# Autodesk Inventor assembly: Robot Transporter
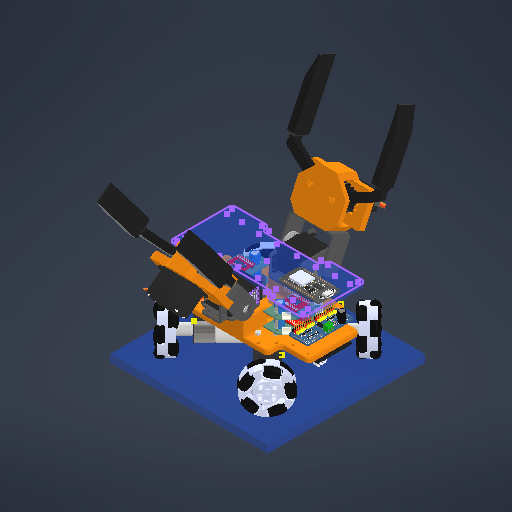
[picture p0: Inventor's stored thumbnail of the model, 512x512]
Saved by Autodesk Inventor 2026.2 (Build 302298000, 298)
## iProperties
Created: 2026-05-17
Part Number: Robot Transporter
Document SubType Name: Assembly
Designer: hando
Author: hando
## Documents named in this file (21)
- D:\Data_Lokal\Kuliah\Tri Wahyu (22518241023)\Lomba Technocorner UGM\02_Transporter\Design Robot\00_Inventor_Workspace\Robot Transporter.iam
- D:\Data_Lokal\Kuliah\Tri Wahyu (22518241023)\Lomba Technocorner UGM\02_Transporter\Design Robot\00_Inventor_Workspace\bringsmart-jga25-371-12v-dc-geared-motor-with-encoder-collection-1.snapshot.3\JGA25-371_12VDC_400RPM.ipt
- D:\Data_Lokal\Kuliah\Tri Wahyu (22518241023)\Lomba Technocorner UGM\02_Transporter\Design Robot\00_Inventor_Workspace\Base.ipt
- D:\Data_Lokal\Kuliah\Tri Wahyu (22518241023)\Lomba Technocorner UGM\02_Transporter\Design Robot\00_Inventor_Workspace\Batas Robot.ipt
- D:\Data_Lokal\Kuliah\Tri Wahyu (22518241023)\Lomba Technocorner UGM\02_Transporter\Design Robot\00_Inventor_Workspace\Roda Omni_53mm.iam
- D:\Data_Lokal\Kuliah\Tri Wahyu (22518241023)\Lomba Technocorner UGM\02_Transporter\Design Robot\00_Inventor_Workspace\motor-dc-servo-gm25-370-gearmotor-1.snapshot.4\PASS DC SERVO GM 25-370 GEAR MOTOR\PASS DC SERVO GM 25-370 GEAR MOT.ipt
- D:\Data_Lokal\Kuliah\Tri Wahyu (22518241023)\Lomba Technocorner UGM\02_Transporter\Design Robot\00_Inventor_Workspace\Hex Coupling\Hex Coupling D4 Mecanum.ipt
- D:\Data_Lokal\Kuliah\Tri Wahyu (22518241023)\Lomba Technocorner UGM\02_Transporter\Design Robot\00_Inventor_Workspace\Assembly1.iam
- D:\Data_Lokal\Kuliah\Tri Wahyu (22518241023)\Lomba Technocorner UGM\02_Transporter\Design Robot\00_Inventor_Workspace\m3-nut-4.snapshot.1\M3 Nut\M3 Nut\M3 Nut.ipt
- D:\Data_Lokal\Kuliah\Tri Wahyu (22518241023)\Lomba Technocorner UGM\02_Transporter\Design Robot\00_Inventor_Workspace\mg996r-servo-motor-3.snapshot.16\MG996R Servo Motor\MG996R Servo Motor\MG996R Servo Motor\MG996R Servo Motor.iam
- D:\Data_Lokal\Kuliah\Tri Wahyu (22518241023)\Lomba Technocorner UGM\02_Transporter\Design Robot\00_Inventor_Workspace\m3-standoff-pcb-spacers-1.snapshot.2\M3_M_TO_F_15MM_STANDOFF\M3_M_TO_F_15MM_STANDOFF\M3_M_TO.ipt
- D:\Data_Lokal\Kuliah\Tri Wahyu (22518241023)\Lomba Technocorner UGM\02_Transporter\Design Robot\00_Inventor_Workspace\Holder_StepDown.ipt
- D:\Data_Lokal\Kuliah\Tri Wahyu (22518241023)\Lomba Technocorner UGM\02_Transporter\Design Robot\00_Inventor_Workspace\pca9685-8.snapshot.1\pca9685\pca9685\pca9685.iam
- D:\Data_Lokal\Kuliah\Tri Wahyu (22518241023)\Lomba Technocorner UGM\02_Transporter\Design Robot\00_Inventor_Workspace\Components\SY8205_Servo_Stepdown_5V5A\SY8205_Servo_Stepdown_5V5A.ipt
- D:\Data_Lokal\Kuliah\Tri Wahyu (22518241023)\Lomba Technocorner UGM\02_Transporter\Design Robot\00_Inventor_Workspace\b2b-jst-xh-90-degree-connector-generic-1.snapshot.3\CONECTOR-2\WHITE\WHITE JST XH 3 PIN CONN.ipt
- D:\Data_Lokal\Kuliah\Tri Wahyu (22518241023)\Lomba Technocorner UGM\02_Transporter\Design Robot\00_Inventor_Workspace\servo-brackets-2.snapshot.3\Multi Purpose Bracket\Multi Purpose Bracket\Multi Purpose Bracket.ipt
- D:\Data_Lokal\Kuliah\Tri Wahyu (22518241023)\Lomba Technocorner UGM\02_Transporter\Design Robot\00_Inventor_Workspace\Wahyu Gripper MG996R\Gripper MG996R.iam
- D:\Data_Lokal\Kuliah\Tri Wahyu (22518241023)\Lomba Technocorner UGM\02_Transporter\Design Robot\00_Inventor_Workspace\servo-brackets-2.snapshot.3\U Bracket\U Bracket\U Bracket.ipt
- D:\Data_Lokal\Kuliah\Tri Wahyu (22518241023)\Lomba Technocorner UGM\02_Transporter\Design Robot\00_Inventor_Workspace\servo-horn-round-for-55g-servo-25t-spline-1.snapshot.1\Servo horn v2\Servo horn v2\Servo horn v2.ipt
- D:\Data_Lokal\Kuliah\Tri Wahyu (22518241023)\Lomba Technocorner UGM\02_Transporter\Design Robot\00_Inventor_Workspace\m3-standoff-pcb-spacers-1.snapshot.2\M3_M_TO_F_20MM_STANDOFF\M3_M_TO_F_20MM_STANDOFF\M3_M_TO.ipt
- D:\Data_Lokal\Kuliah\Tri Wahyu (22518241023)\Lomba Technocorner UGM\02_Transporter\Design Robot\00_Inventor_Workspace\esp32_30pin\esp32_30pin.iam
## Components (49 placed, 19 different names)
1. JGA25-371_12VDC_400RPM:1 — Mate:82, Mate:84, Mate:108, Flush:33
2. Base:1 — Flush:1, Flush:2, Mate:83, Mate:89, Mate:91, Mate:92, Mate:94, Mate:96, Mate:97, Mate:98, Mate:99, Mate:100, Mate:103, Mate:104, Mate:105, Flush:32, Flush:33, Flush:35, Flush:36, Mate:133, Mate:134, Mate:135, Mate:137, Mate:142, Mate:143, Mate:148, Mate:216, Flush:182, Flush:183, Mate:235, Flush:185, Mate:236, Flush:186, Flush:187, Flush:188, Mate:247, Mate:248, Mate:250, Mate:262, Mate:263, Mate:265, Mate:266, Mate:267
3. JGA25-371_12VDC_400RPM:2 — Mate:101, Mate:102, Mate:106, Flush:35
4. JGA25-371_12VDC_400RPM:3 — Mate:93, Mate:95, Mate:111, Flush:32
5. JGA25-371_12VDC_400RPM:4 — Mate:114, Mate:115, Mate:116, Flush:36
6. Batas Robot:1 — Flush:1, Flush:2, Mate:89
7. Roda Omni_53mm:1 [sub-assembly] — Mate:113, Mate:123
8. Roda Omni_53mm:2 [sub-assembly] — Mate:88, Mate:122
9. Roda Omni_53mm:3 [sub-assembly] — Mate:118, Mate:125
10. Roda Omni_53mm:4 [sub-assembly] — Mate:110, Mate:124
11. PASS DC SERVO GM 25-370 GEAR MOT:1 — Mate:82, Mate:83, Mate:84, Mate:96, Mate:97, Mate:107
12. Hex Coupling D4 Mecanum:1 — Mate:88, Mate:107, Mate:108, Mate:122
13. PASS DC SERVO GM 25-370 GEAR MOT:2 — Mate:91, Mate:92, Mate:93, Mate:94, Mate:95, Mate:112
14. PASS DC SERVO GM 25-370 GEAR MOT:3 — Mate:98, Mate:99, Mate:100, Mate:101, Mate:102, Mate:109
15. PASS DC SERVO GM 25-370 GEAR MOT:4 — Mate:103, Mate:104, Mate:105, Mate:114, Mate:115, Mate:117
16. Hex Coupling D4 Mecanum:2 — Mate:106, Mate:109, Mate:110, Mate:124
17. Hex Coupling D4 Mecanum:3 — Mate:111, Mate:112, Mate:113, Mate:123
18. Hex Coupling D4 Mecanum:4 — Mate:116, Mate:117, Mate:118, Mate:125
19. Assembly1:1 [sub-assembly] — Mate:227, Mate:229, Mate:231
20. Assembly1:2 [sub-assembly] — Mate:217, Mate:235, Flush:185, Mate:239, Mate:240, Mate:241
21. Assembly1:3 [sub-assembly] — Mate:239, Mate:240, Mate:242, Mate:244, Mate:245
22. Assembly1:4 [sub-assembly] — Mate:223, Flush:182, Mate:224, Mate:225, Mate:226
23. M3 Nut:1 — Mate:133, Mate:134
24. M3 Nut:2 — Mate:135, Mate:137, Mate:223, Mate:224
25. M3 Nut:4 — Mate:142, Mate:143
26. M3 Nut:5 — Mate:148, Mate:216, Mate:217
27. MG996R Servo Motor:1 [sub-assembly] — Mate:206, Mate:207, Mate:249, Flush:190, Mate:251
28. M3_M_TO:4 — Mate:225, Mate:226, Mate:227, Mate:229, Mate:230
29. M3_M_TO:5 — Mate:236, Mate:238, Mate:241, Mate:243
30. Holder_StepDown:1 — Flush:183, Flush:188, Flush:189, Mate:246
31. pca9685:1 [sub-assembly] — Flush:186, Flush:187
32. SY8205_Servo_Stepdown_5V5A:1 — Mate:202, Flush:175, Flush:176, Mate:267
33. SY8205_Servo_Stepdown_5V5A:2 — Mate:201, Flush:173, Flush:174, Mate:266
34. SY8205_Servo_Stepdown_5V5A:3
35. WHITE JST XH 3 PIN CONN:1 — Mate:201, Flush:173, Flush:174
36. WHITE JST XH 3 PIN CONN:2 — Mate:202, Flush:175, Flush:176
37. Multi Purpose Bracket:1 — Mate:247, Mate:248, Mate:249, Mate:250, Flush:190, Mate:251
38. Gripper MG996R:1 [sub-assembly] — Mate:212, Mate:213, Mate:214
39. U Bracket:1 — Mate:208, Mate:209, Mate:210, Mate:212, Mate:213, Mate:214
40. Servo horn v2:1 — Mate:206, Mate:207, Mate:208, Mate:209, Mate:210
41. M3_M_TO:7 — Mate:230, Mate:231
42. M3_M_TO:8 — Mate:244, Mate:245
43. M3 Nut:6 — Mate:238, Mate:242, Mate:243
44. esp32_30pin:1 [sub-assembly] — Flush:189, Mate:246
45. MG996R Servo Motor:2 [sub-assembly] — Mate:264
46. Multi Purpose Bracket:2 — Mate:262, Mate:263, Mate:264, Mate:265
47. Gripper MG996R:2 [sub-assembly]
48. U Bracket:2
49. Servo horn v2:2
## Relationships (114: Mate 95, Flush 19)
- Flush:1 (50 mm): Base:1 ↔ Batas Robot:1
- Flush:2 (50 mm): Base:1 ↔ Batas Robot:1
- Mate:82: JGA25-371_12VDC_400RPM:1 ↔ PASS DC SERVO GM 25-370 GEAR MOT:1
- Mate:83: Base:1 ↔ PASS DC SERVO GM 25-370 GEAR MOT:1
- Mate:84: JGA25-371_12VDC_400RPM:1 ↔ PASS DC SERVO GM 25-370 GEAR MOT:1
- Mate:88: Roda Omni_53mm:2 ↔ Hex Coupling D4 Mecanum:1
- Mate:89 (47 mm): Base:1 ↔ Batas Robot:1
- Mate:91: Base:1 ↔ PASS DC SERVO GM 25-370 GEAR MOT:2
- Mate:92: Base:1 ↔ PASS DC SERVO GM 25-370 GEAR MOT:2
- Mate:93: JGA25-371_12VDC_400RPM:3 ↔ PASS DC SERVO GM 25-370 GEAR MOT:2
- Mate:94: Base:1 ↔ PASS DC SERVO GM 25-370 GEAR MOT:2
- Mate:95: JGA25-371_12VDC_400RPM:3 ↔ PASS DC SERVO GM 25-370 GEAR MOT:2
- Mate:96: Base:1 ↔ PASS DC SERVO GM 25-370 GEAR MOT:1
- Mate:97: Base:1 ↔ PASS DC SERVO GM 25-370 GEAR MOT:1
- Mate:98: Base:1 ↔ PASS DC SERVO GM 25-370 GEAR MOT:3
- Mate:99: Base:1 ↔ PASS DC SERVO GM 25-370 GEAR MOT:3
- Mate:100: Base:1 ↔ PASS DC SERVO GM 25-370 GEAR MOT:3
- Mate:101: JGA25-371_12VDC_400RPM:2 ↔ PASS DC SERVO GM 25-370 GEAR MOT:3
- Mate:102: JGA25-371_12VDC_400RPM:2 ↔ PASS DC SERVO GM 25-370 GEAR MOT:3
- Mate:103: Base:1 ↔ PASS DC SERVO GM 25-370 GEAR MOT:4
- Mate:104: Base:1 ↔ PASS DC SERVO GM 25-370 GEAR MOT:4
- Mate:105: Base:1 ↔ PASS DC SERVO GM 25-370 GEAR MOT:4
- Mate:106: JGA25-371_12VDC_400RPM:2 ↔ Hex Coupling D4 Mecanum:2
- Mate:107: PASS DC SERVO GM 25-370 GEAR MOT:1 ↔ Hex Coupling D4 Mecanum:1
- Mate:108: JGA25-371_12VDC_400RPM:1 ↔ Hex Coupling D4 Mecanum:1
- Mate:109: PASS DC SERVO GM 25-370 GEAR MOT:3 ↔ Hex Coupling D4 Mecanum:2
- Mate:110: Roda Omni_53mm:4 ↔ Hex Coupling D4 Mecanum:2
- Mate:111: JGA25-371_12VDC_400RPM:3 ↔ Hex Coupling D4 Mecanum:3
- Mate:112: PASS DC SERVO GM 25-370 GEAR MOT:2 ↔ Hex Coupling D4 Mecanum:3
- Mate:113: Roda Omni_53mm:1 ↔ Hex Coupling D4 Mecanum:3
- Mate:114: JGA25-371_12VDC_400RPM:4 ↔ PASS DC SERVO GM 25-370 GEAR MOT:4
- Mate:115: JGA25-371_12VDC_400RPM:4 ↔ PASS DC SERVO GM 25-370 GEAR MOT:4
- Flush:32: Base:1 ↔ JGA25-371_12VDC_400RPM:3
- Flush:33: JGA25-371_12VDC_400RPM:1 ↔ Base:1
- Mate:116: JGA25-371_12VDC_400RPM:4 ↔ Hex Coupling D4 Mecanum:4
- Mate:117: PASS DC SERVO GM 25-370 GEAR MOT:4 ↔ Hex Coupling D4 Mecanum:4
- Mate:118: Roda Omni_53mm:3 ↔ Hex Coupling D4 Mecanum:4
- Flush:35: Base:1 ↔ JGA25-371_12VDC_400RPM:2
- Flush:36: Base:1 ↔ JGA25-371_12VDC_400RPM:4
- Mate:122: Roda Omni_53mm:2 ↔ Hex Coupling D4 Mecanum:1
- Mate:123: Roda Omni_53mm:1 ↔ Hex Coupling D4 Mecanum:3
- Mate:124: Roda Omni_53mm:4 ↔ Hex Coupling D4 Mecanum:2
- Mate:125: Roda Omni_53mm:3 ↔ Hex Coupling D4 Mecanum:4
- Mate:133: Base:1 ↔ M3 Nut:1
- Mate:134: Base:1 ↔ M3 Nut:1
- Mate:135: Base:1 ↔ M3 Nut:2
- Mate:137: Base:1 ↔ M3 Nut:2
- Mate:142: Base:1 ↔ M3 Nut:4
- Mate:143: Base:1 ↔ M3 Nut:4
- Mate:148: Base:1 ↔ M3 Nut:5
- Mate:201: SY8205_Servo_Stepdown_5V5A:2 ↔ WHITE JST XH 3 PIN CONN:1
- Flush:173 (0.4 mm): SY8205_Servo_Stepdown_5V5A:2 ↔ WHITE JST XH 3 PIN CONN:1
- Flush:174 (0.4 mm): SY8205_Servo_Stepdown_5V5A:2 ↔ WHITE JST XH 3 PIN CONN:1
- Mate:202: SY8205_Servo_Stepdown_5V5A:1 ↔ WHITE JST XH 3 PIN CONN:2
- Flush:175 (0.4 mm): SY8205_Servo_Stepdown_5V5A:1 ↔ WHITE JST XH 3 PIN CONN:2
- Flush:176 (0.4 mm): SY8205_Servo_Stepdown_5V5A:1 ↔ WHITE JST XH 3 PIN CONN:2
- Mate:206: MG996R Servo Motor:1 ↔ Servo horn v2:1
- Mate:207: MG996R Servo Motor:1 ↔ Servo horn v2:1
- Mate:208: U Bracket:1 ↔ Servo horn v2:1
- Mate:209: U Bracket:1 ↔ Servo horn v2:1
- Mate:210: U Bracket:1 ↔ Servo horn v2:1
- Mate:212: Gripper MG996R:1 ↔ U Bracket:1
- Mate:213: Gripper MG996R:1 ↔ U Bracket:1
- Mate:214: Gripper MG996R:1 ↔ U Bracket:1
- Mate:216: Base:1 ↔ M3 Nut:5
- Mate:217: Assembly1:2 ↔ M3 Nut:5
- Mate:223: Assembly1:4 ↔ M3 Nut:2
- Flush:182: Base:1 ↔ Assembly1:4
- Mate:224: Assembly1:4 ↔ M3 Nut:2
- Mate:225: Assembly1:4 ↔ M3_M_TO:4
- Mate:226: Assembly1:4 ↔ M3_M_TO:4
- Mate:227: Assembly1:1 ↔ M3_M_TO:4
- Mate:229: Assembly1:1 ↔ M3_M_TO:4
- Mate:230: M3_M_TO:4 ↔ M3_M_TO:7
- Mate:231: Assembly1:1 ↔ M3_M_TO:7
- Flush:183 (10 mm): Base:1 ↔ Holder_StepDown:1
- Mate:235: Base:1 ↔ Assembly1:2
- Flush:185: Base:1 ↔ Assembly1:2
- Mate:236: Base:1 ↔ M3_M_TO:5
- Mate:238: M3_M_TO:5 ↔ M3 Nut:6
- Mate:239: Assembly1:2 ↔ Assembly1:3
- Mate:240: Assembly1:2 ↔ Assembly1:3
- Mate:241: Assembly1:2 ↔ M3_M_TO:5
- Mate:242: Assembly1:3 ↔ M3 Nut:6
- Mate:243: M3_M_TO:5 ↔ M3 Nut:6
- Mate:244: Assembly1:3 ↔ M3_M_TO:8
- Mate:245: Assembly1:3 ↔ M3_M_TO:8
- Flush:186 (2.5 mm): Base:1 ↔ pca9685:1
- Flush:187 (4 mm): Base:1 ↔ pca9685:1
- Flush:188: Base:1 ↔ Holder_StepDown:1
- Flush:189 (5 mm): Holder_StepDown:1 ↔ esp32_30pin:1
- Mate:246: Holder_StepDown:1 ↔ esp32_30pin:1
- Mate:247: Base:1 ↔ Multi Purpose Bracket:1
- Mate:248: Base:1 ↔ Multi Purpose Bracket:1
- Mate:249: MG996R Servo Motor:1 ↔ Multi Purpose Bracket:1
- Mate:250: Base:1 ↔ Multi Purpose Bracket:1
- Flush:190: MG996R Servo Motor:1 ↔ Multi Purpose Bracket:1
- Mate:251: MG996R Servo Motor:1 ↔ Multi Purpose Bracket:1
- [Mate]: MG996R Servo Motor:2 ↔ Servo horn v2:2
- [Mate]: MG996R Servo Motor:2 ↔ Servo horn v2:2
- [Mate]: U Bracket:2 ↔ Servo horn v2:2
- [Mate]: U Bracket:2 ↔ Servo horn v2:2
- [Mate]: U Bracket:2 ↔ Servo horn v2:2
- [Mate]: Gripper MG996R:2 ↔ U Bracket:2
- [Mate]: Gripper MG996R:2 ↔ U Bracket:2
- [Mate]: Gripper MG996R:2 ↔ U Bracket:2
- [Flush]: MG996R Servo Motor:2 ↔ Multi Purpose Bracket:2
- [Mate]: MG996R Servo Motor:2 ↔ Multi Purpose Bracket:2
- Mate:262: Base:1 ↔ Multi Purpose Bracket:2
- Mate:263: Base:1 ↔ Multi Purpose Bracket:2
- Mate:264: MG996R Servo Motor:2 ↔ Multi Purpose Bracket:2
- Mate:265: Base:1 ↔ Multi Purpose Bracket:2
- Mate:266: Base:1 ↔ SY8205_Servo_Stepdown_5V5A:2
- Mate:267: Base:1 ↔ SY8205_Servo_Stepdown_5V5A:1
## Named parameters: d553_d548 = 0 mm, d554_d549 = 0 mm, d555_d550 = 0 mm, d556_d551 = 0 mm, d557_d458 = 0 mm, d558_d459 = 0 mm, d559_d460 = 0 mm, d560_d463 = 0 mm, d561_d464 = 0 mm, d562_d466 = 0 mm, d563_d471 = 0 mm, d564_d472 = 0 mm
